# Autodesk Inventor assembly: carbide_probe_insulated_20deg_tip_r01
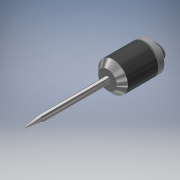
[picture p0: Inventor's stored thumbnail of the model, 180x180]
Saved by Autodesk Inventor 2016 (Build 200138000, 138)
## iProperties
Created: 2017-01-09
Part Number: carbide_probe_insulated_20deg_tip_r01
Document SubType Name: Assembly
Designer: Valued Customer
Author: Valued Customer
## Documents named in this file (4)
- C:\fly-design-files\antenna-probes\carbide_probe_insulated_20deg_tip_r01\carbide_probe_insulated_20deg_tip_r01.iam
- C:\fly-design-files\antenna-probes\carbide_probe_insulated_20deg_tip_r01\carbide_probe_insulated_20deg_tip_r01.ipt
- C:\fly-design-files\antenna-probes\carbide_probe_insulated_20deg_tip_r01\threaded_rod_m3_x05_6mm_r01.ipt
- C:\fly-design-files\antenna-probes\carbide_probe_insulated_20deg_tip_r01\washer_m3_r01.ipt
## Components (3 placed, 3 different names)
1. carbide_probe_insulated_20deg_tip_r01:1 — Insert:1, Insert:2
2. threaded_rod_m3_x05_6mm_r01:1 — Insert:1
3. washer_m3_r01:1 — Insert:2
## Relationships (2: Insert 2)
- Insert:1: carbide_probe_insulated_20deg_tip_r01:1 ↔ threaded_rod_m3_x05_6mm_r01:1
- Insert:2: carbide_probe_insulated_20deg_tip_r01:1 ↔ washer_m3_r01:1
